# Autodesk Inventor assembly: step 1b
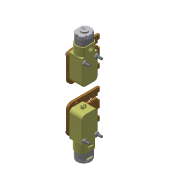
[picture p0: Inventor's stored thumbnail of the model, 180x180]
Saved by Autodesk Inventor 2016 (Build 200138000, 138)
## iProperties
Created: 2015-07-07
Part Number: step 1b
Document SubType Name: Assembly
Designer: Sebastian
Author: Sebastian
## Documents named in this file (3)
- C:\Users\Sebastian\Desktop\step 1b.iam
- D:\Unsorted\29-01-2015\Sebastian\Documents\Inventor\ERNIE\motor mount - right.iam
- D:\Unsorted\29-01-2015\Sebastian\Documents\Inventor\ERNIE\motor mount.iam
## Components (2 placed, 2 different names)
1. motor mount - right:1 [sub-assembly] — Flush:1, Flush:2
2. motor mount:1 [sub-assembly] — Flush:1, Flush:2
## Relationships (2: Flush 2)
- Flush:1: motor mount - right:1 ↔ motor mount:1
- Flush:2: motor mount - right:1 ↔ motor mount:1
